# Autodesk Inventor assembly: EstanteColgado
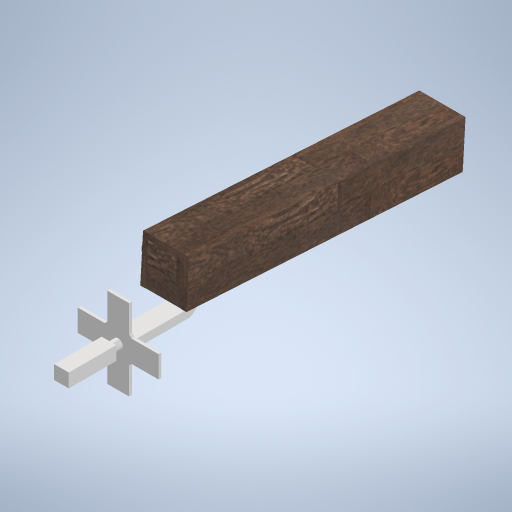
[picture p0: Inventor's stored thumbnail of the model, 512x512]
Saved by Autodesk Inventor 2023 (Build 270158000, 158)
## iProperties
Created: 2023-05-30
Part Number: EstanteColgado
Document SubType Name: Assembly
Designer: WIN10
Author: WIN10
## Documents named in this file (3)
- C:\Users\WIN10\DisenoDeProduccion\ModelosCeldaRobotica\EstanteColgado.iam
- C:\Users\WIN10\DisenoDeProduccion\ModelosCeldaRobotica\Gancho.ipt
- C:\Users\WIN10\Downloads\RepisaLego.iam
## Components (2 placed, 2 different names)
1. Gancho:1 — Coincidencia:2, Coincidencia:3, Coincidencia:4, Coincidencia:6, Coincidencia:7
2. RepisaLego:1 [sub-assembly] — Coincidencia:6, Coincidencia:7
## Relationships (5: Mate 5)
- Coincidencia:2 [Mate]: Gancho:1
- Coincidencia:3 [Mate]: Gancho:1
- Coincidencia:4 [Mate]: Gancho:1
- Coincidencia:6 [Mate]: Gancho:1 ↔ RepisaLego:1
- Coincidencia:7 [Mate]: Gancho:1 ↔ RepisaLego:1
